# Autodesk Inventor assembly: Cube 1x1 V5 (Sample)
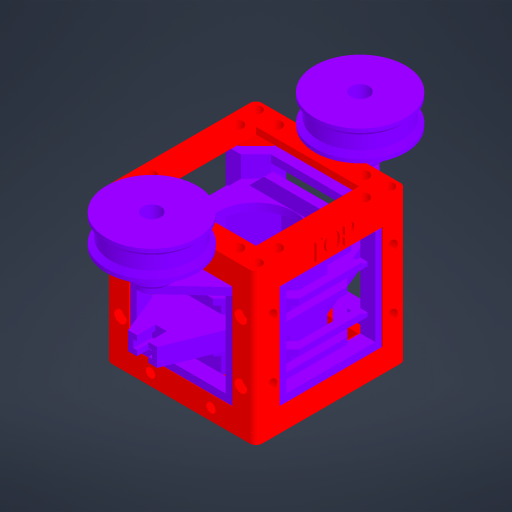
[picture p0: Inventor's stored thumbnail of the model, 512x512]
Saved by Autodesk Inventor 2023.4 (Build 274418000, 418)
## iProperties
Created: 2022-08-13
Part Number: Cube 1x1 V5 (Sample)
Document SubType Name: Assembly
Designer: xSibe
Author: xSibe
## Documents named in this file (4)
- C:\.Laptop\.Work\Projects\Project Protocube\1 Autodesk\1 Cubes\Sample\Cube 1x1 V5 (Sample).iam
- C:\.Laptop\.Work\Projects\Project Protocube\1 Autodesk\1 Cubes\Sample\Z Axis Sample V1.ipt
- C:\.Laptop\.Work\Projects\Project Protocube\1 Autodesk\1 Cubes\Sample\Z Axis Handle.ipt
- C:\.Laptop\.Work\Projects\Project Protocube\1 Autodesk\1 Cubes\Cubes\Cube 1x1 V5.iam
## Components (4 placed, 3 different names)
1. Z Axis Sample V1:1 — Mate:4, Mate:5, Mate:10, Mate:11, Mate:12, Mate:13
2. Z Axis Handle:1 — Mate:10, Mate:13
3. Z Axis Handle:2 — Mate:11, Mate:12
4. Cube 1x1 V5:1 [sub-assembly]
## Relationships (6: Mate 6)
- Mate:4: Z Axis Sample V1:1
- Mate:5: Z Axis Sample V1:1
- Mate:10: Z Axis Sample V1:1 ↔ Z Axis Handle:1
- Mate:11: Z Axis Sample V1:1 ↔ Z Axis Handle:2
- Mate:12: Z Axis Sample V1:1 ↔ Z Axis Handle:2
- Mate:13: Z Axis Sample V1:1 ↔ Z Axis Handle:1
